# Autodesk Inventor assembly: Assembly1
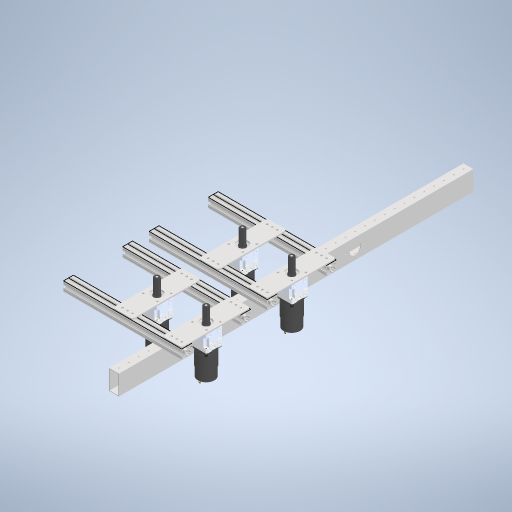
[picture p0: Inventor's stored thumbnail of the model, 512x512]
Saved by Autodesk Inventor 2024 (Build 280153000, 153)
## iProperties
Created: 2023-08-12
Part Number: Assembly1
Document SubType Name: Assembly
Designer: Gabriel Marquez
Author: Gabriel Marquez
## Documents named in this file (5)
- C:\Users\Gabriel Marquez\OneDrive\Documents\GitHub\T3-CAD\Current Season CAD\Body\Assembly1.iam
- C:\Users\Gabriel Marquez\OneDrive\Documents\GitHub\T3-CAD\Current Season CAD\Body\gun turret main spar.ipt
- C:\Users\Gabriel Marquez\OneDrive\Documents\GitHub\T3-CAD\Current Season CAD\Body\Shooter Sliding Motor Mount Plate V1.1.ipt
- C:\Users\Gabriel Marquez\OneDrive\Documents\GitHub\T3-CAD\Current Season CAD\Body\T channel for shooter.ipt
- C:\Users\Gabriel Marquez\OneDrive\Documents\GitHub\T3-CAD\Stock\Motors and Gearboxes\VersaPlanetary v2 Single Stage 10_1 with 775 Series  (1)\VersaPlanetary v2 Single Stage 10_1 with 775 Series  (1).iam
## Components (13 placed, 4 different names)
1. gun turret main spar:1 — Mate:11, Mate:12, Flush:4, Flush:8, Flush:9, Mate:23
2. Shooter Sliding Motor Mount Plate V1.1:1 — Mate:1, Mate:2, Flush:1, Mate:3, Mate:4, Flush:2, Rotational:1, Rotational:2
3. T channel for shooter:1 — Mate:1, Mate:2, Flush:1, Mate:5, Mate:6, Flush:3, Mate:11, Flush:4
4. T channel for shooter:4 — Mate:3, Mate:4, Flush:2, Mate:7, Mate:8, Mate:12
5. Shooter Sliding Motor Mount Plate V1.1:2 — Mate:5, Mate:6, Mate:7, Mate:8, Flush:3, Mate:9, Mate:10, Mate:27
6. VersaPlanetary v2 Single Stage 10_1 with 775 Series  (1):1 [sub-assembly] — Rotational:1, Rotational:2
7. VersaPlanetary v2 Single Stage 10_1 with 775 Series  (1):2 [sub-assembly] — Mate:9, Mate:10, Mate:27
8. Shooter Sliding Motor Mount Plate V1.1:3 — Mate:24, Mate:25
9. T channel for shooter:5 — Flush:8, Mate:23, Mate:24
10. T channel for shooter:6 — Flush:9, Mate:25
11. Shooter Sliding Motor Mount Plate V1.1:4 — Mate:26
12. VersaPlanetary v2 Single Stage 10_1 with 775 Series  (1):3 [sub-assembly]
13. VersaPlanetary v2 Single Stage 10_1 with 775 Series  (1):4 [sub-assembly] — Mate:26
## Relationships (40: Mate 27, Flush 9, RevoluteJoint 4)
- Mate:1: Shooter Sliding Motor Mount Plate V1.1:1 ↔ T channel for shooter:1
- Mate:2: Shooter Sliding Motor Mount Plate V1.1:1 ↔ T channel for shooter:1
- Flush:1: Shooter Sliding Motor Mount Plate V1.1:1 ↔ T channel for shooter:1
- Mate:3: Shooter Sliding Motor Mount Plate V1.1:1 ↔ T channel for shooter:4
- Mate:4: Shooter Sliding Motor Mount Plate V1.1:1 ↔ T channel for shooter:4
- Flush:2: Shooter Sliding Motor Mount Plate V1.1:1 ↔ T channel for shooter:4
- Mate:5: T channel for shooter:1 ↔ Shooter Sliding Motor Mount Plate V1.1:2
- Mate:6: T channel for shooter:1 ↔ Shooter Sliding Motor Mount Plate V1.1:2
- Mate:7: T channel for shooter:4 ↔ Shooter Sliding Motor Mount Plate V1.1:2
- Mate:8: T channel for shooter:4 ↔ Shooter Sliding Motor Mount Plate V1.1:2
- Flush:3 (127 mm): T channel for shooter:1 ↔ Shooter Sliding Motor Mount Plate V1.1:2
- Rotational:1 [RevoluteJoint]: Shooter Sliding Motor Mount Plate V1.1:1 ↔ VersaPlanetary v2 Single Stage 10_1 with 775 Series  (1):1
- Rotational:2 [RevoluteJoint]: Shooter Sliding Motor Mount Plate V1.1:1 ↔ VersaPlanetary v2 Single Stage 10_1 with 775 Series  (1):1
- Mate:9: Shooter Sliding Motor Mount Plate V1.1:2 ↔ VersaPlanetary v2 Single Stage 10_1 with 775 Series  (1):2
- Mate:10: Shooter Sliding Motor Mount Plate V1.1:2 ↔ VersaPlanetary v2 Single Stage 10_1 with 775 Series  (1):2
- Mate:11: gun turret main spar:1 ↔ T channel for shooter:1
- Mate:12: gun turret main spar:1 ↔ T channel for shooter:4
- Flush:4 (50.8 mm): gun turret main spar:1 ↔ T channel for shooter:1
- [Mate]: Shooter Sliding Motor Mount Plate V1.1:3 ↔ T channel for shooter:5
- [Mate]: Shooter Sliding Motor Mount Plate V1.1:3 ↔ T channel for shooter:5
- [Flush]: Shooter Sliding Motor Mount Plate V1.1:3 ↔ T channel for shooter:5
- [Mate]: Shooter Sliding Motor Mount Plate V1.1:3 ↔ T channel for shooter:6
- [Mate]: Shooter Sliding Motor Mount Plate V1.1:3 ↔ T channel for shooter:6
- [Flush]: Shooter Sliding Motor Mount Plate V1.1:3 ↔ T channel for shooter:6
- [Mate]: T channel for shooter:5 ↔ Shooter Sliding Motor Mount Plate V1.1:4
- [Mate]: T channel for shooter:5 ↔ Shooter Sliding Motor Mount Plate V1.1:4
- [Mate]: T channel for shooter:6 ↔ Shooter Sliding Motor Mount Plate V1.1:4
- [Mate]: T channel for shooter:6 ↔ Shooter Sliding Motor Mount Plate V1.1:4
- [Flush] (127 mm): T channel for shooter:5 ↔ Shooter Sliding Motor Mount Plate V1.1:4
- [RevoluteJoint]: Shooter Sliding Motor Mount Plate V1.1:3 ↔ VersaPlanetary v2 Single Stage 10_1 with 775 Series  (1):3
- [RevoluteJoint]: Shooter Sliding Motor Mount Plate V1.1:3 ↔ VersaPlanetary v2 Single Stage 10_1 with 775 Series  (1):3
- [Mate]: Shooter Sliding Motor Mount Plate V1.1:4 ↔ VersaPlanetary v2 Single Stage 10_1 with 775 Series  (1):4
- [Mate]: Shooter Sliding Motor Mount Plate V1.1:4 ↔ VersaPlanetary v2 Single Stage 10_1 with 775 Series  (1):4
- Flush:8 (50.8 mm): gun turret main spar:1 ↔ T channel for shooter:5
- Flush:9 (50.8 mm): gun turret main spar:1 ↔ T channel for shooter:6
- Mate:23: gun turret main spar:1 ↔ T channel for shooter:5
- Mate:24: Shooter Sliding Motor Mount Plate V1.1:3 ↔ T channel for shooter:5
- Mate:25: Shooter Sliding Motor Mount Plate V1.1:3 ↔ T channel for shooter:6
- Mate:26: Shooter Sliding Motor Mount Plate V1.1:4 ↔ VersaPlanetary v2 Single Stage 10_1 with 775 Series  (1):4
- Mate:27: Shooter Sliding Motor Mount Plate V1.1:2 ↔ VersaPlanetary v2 Single Stage 10_1 with 775 Series  (1):2
## Named parameters: d20_d0 = 0 mm, d21_d1 = 0 mm, d22_d2 = 0 mm, d23_d3 = 0 mm, d24_d4 = 0 mm, d25_d5 = 0 mm, d26_d6 = 0 mm, d27_d7 = 0 mm, d28_d8 = 0 mm, d29_d9 = 0 mm, d30_d10 = 127 mm, d31_d11 = 0 mm, d32_d12 = 135 deg, d33_d13 = 0 mm, d34_d14 = -135 deg, d35_d15 = 0 mm, d36_d16 = 0 mm
